# Autodesk Inventor assembly: segment2
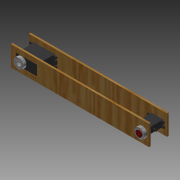
[picture p0: Inventor's stored thumbnail of the model, 180x180]
Saved by Autodesk Inventor 2013 (Build 170138000, 138)
## iProperties
Created: 2014-10-10
Part Number: segment2
Document SubType Name: Assembly
Designer: Masta
Mass: 122.392 g
Surface Area: 538.403 cm^2
Volume: 141.928 cm^3
Density: 0.862349 g/cm^3
Author: Masta
## Documents named in this file (7)
- D:\DrOctopus\3D model\arm\segment2.iam
- D:\DrOctopus\3D model\arm\servo 13kg BMS-630MG.ipt
- D:\DrOctopus\3D model\arm\segment2a.ipt
- D:\DrOctopus\3D model\arm\serwo 2.8kg DS939HV.ipt
- D:\DrOctopus\3D model\arm\Bearing 699ZZ - 9x20x6mm.ipt
- D:\DrOctopus\3D model\arm\segment2b.ipt
- D:\DrOctopus\3D model\arm\segment1_coupler1.ipt
## Components (7 placed, 6 different names)
1. servo 13kg BMS-630MG:1 — Insert:4, Insert:5, Mate:2, Mate:3
2. segment2a:2 — Insert:4, Insert:5, Insert:6, Insert:7, Insert:8, Flush:1
3. serwo 2.8kg DS939HV:1 — Insert:6, Insert:7
4. Bearing 699ZZ - 9x20x6mm:1 — Mate:2, Mate:3
5. Bearing 699ZZ - 9x20x6mm:2 — Insert:9, Insert:10
6. segment2b:1 — Insert:8, Flush:1, Insert:9
7. segment1_coupler1:1 — Insert:10
## Relationships (10: Insert 7, Mate 2, Flush 1)
- Insert:4 (1 mm): servo 13kg BMS-630MG:1 ↔ segment2a:2
- Insert:5 (1 mm): servo 13kg BMS-630MG:1 ↔ segment2a:2
- Insert:6 (2 mm): segment2a:2 ↔ serwo 2.8kg DS939HV:1
- Insert:7 (2 mm): segment2a:2 ↔ serwo 2.8kg DS939HV:1
- Mate:2: servo 13kg BMS-630MG:1 ↔ Bearing 699ZZ - 9x20x6mm:1
- Mate:3: servo 13kg BMS-630MG:1 ↔ Bearing 699ZZ - 9x20x6mm:1
- Insert:8 (32 mm): segment2a:2 ↔ segment2b:1
- Flush:1: segment2a:2 ↔ segment2b:1
- Insert:9: Bearing 699ZZ - 9x20x6mm:2 ↔ segment2b:1
- Insert:10: Bearing 699ZZ - 9x20x6mm:2 ↔ segment1_coupler1:1
